# Autodesk Inventor assembly: NewChassis
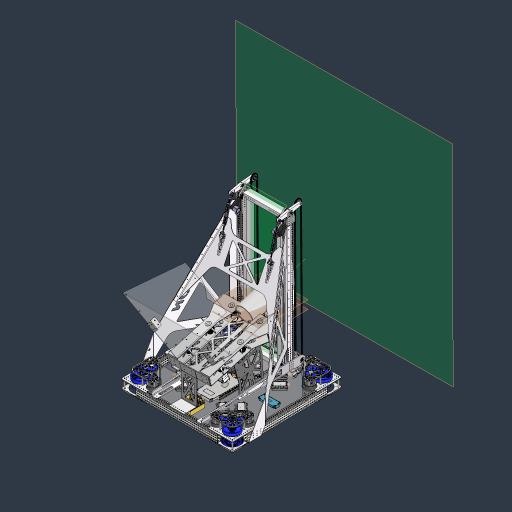
[picture p0: Inventor's stored thumbnail of the model, 512x512]
Saved by Autodesk Inventor 2024.3 (Build 283343000, 343)
## iProperties
ILogicPurgeVersion: 0.0.0.0
OnSaveVersion: 3.4.3.0
OnSaveAssembly: COREAutomationManager
Created: 2025-01-13
Part Number: NewChassis
Document SubType Name: Assembly
Designer: Marcus Tannini
Mfg Approved By: John.Thibert
Mass: 39455.4 g
Surface Area: 111693 cm^2
Volume: 16470.6 cm^3
Density: 2.3955 g/cm^3
ModelCat: Uncategorized
CN_MASS: 40.55
Author: Marcus Tannini
## Documents named in this file (60)
- D:\Inventor Projects\Poseidon V2\#Poseidon 2025.iam
- D:\Inventor Projects\Poseidon V2\ASSY,MK4i,Swerve_Module_INV.iam
- D:\Inventor Projects\Poseidon V2\MAXTube-2x1-Holes.ipt
- D:\Inventor Projects\Poseidon V2\BellyPanTop.ipt
- D:\Inventor Projects\Poseidon V2\BellyPanBot.ipt
- D:\Inventor Projects\Poseidon V2\BATTERY,12V.ipt
- D:\Inventor Projects\Poseidon V2\CONTROLS,MAIN_BREAKER.ipt
- D:\Inventor Projects\Poseidon V2\CONTROLS,MOTOR,NEO,550.ipt
- D:\Inventor Projects\Poseidon V2\CONTROLS,PDH.ipt
- D:\Inventor Projects\Poseidon V2\CONTROLS,PH.ipt
- D:\Inventor Projects\Poseidon V2\CONTROLS,ROBO_RIO.ipt
- D:\Inventor Projects\Poseidon V2\CONTROLS,SPARK_MAX.ipt
- D:\Inventor Projects\Poseidon V2\CONTROLS,VRM.ipt
- D:\Inventor Projects\Poseidon V2\COVER,SPARKMAX.ipt
- D:\Inventor Projects\Poseidon V2\ModifiedCase(IncludesPatterning).iam
- D:\Inventor Projects\Poseidon V2\PLATE,MOUNT,BATTERY,TOP.ipt
- D:\Inventor Projects\Poseidon V2\PLATE,MOUNT,BATTERY,BOT.ipt
- D:\Inventor Projects\Poseidon V2\MOUNT,STRAP,BATTERY.ipt
- D:\Inventor Projects\Poseidon V2\SPACER,SPROCKET,IDLER,ELEVATOR.ipt
- D:\Inventor Projects\Poseidon V2\22.ipt
- D:\Inventor Projects\Poseidon V2\PLATE,MOUNT,DRIVE,ELEVATOR.ipt
- D:\Inventor Projects\Poseidon V2\PLATE,BEARING,DRIVE,ELEVATOR.ipt
- D:\Inventor Projects\Poseidon V2\PURCHASED,HEX_BEARING.ipt
- D:\Inventor Projects\Poseidon V2\SHAFT,HEX,0.500in,DRIVE,ELEVATOR.ipt
- D:\Inventor Projects\Poseidon V2\PLATE,SIDE,BRACE,RIGHT,ELEVATOR.ipt
- D:\Inventor Projects\Poseidon V2\PLATE,SIDE,BRACE,LEFT,ELEVATOR.ipt
- D:\Inventor Projects\Poseidon V2\PLATE,TURNBUCKLE,TENSIONER,CHAIN.ipt
- D:\Inventor Projects\Poseidon V2\PLATE,BRACE,HORISONTAL,TOP,ELEVATOR.ipt
- D:\Inventor Projects\Poseidon V2\TURNBUCKLE,0.25IN_CLEVIS.iam
- D:\Inventor Projects\Poseidon V2\STAGE1,ELEVATOR.iam
- D:\Inventor Projects\Poseidon V2\ASSY,MAIN,ELEVATOR.iam
- D:\Inventor Projects\Poseidon V2\ANGLE,MOUNT,ELEVATOR.ipt
- D:\Inventor Projects\Poseidon V2\ANGLE,MOUNT,ELEVATOR,MIRR.ipt
- D:\Inventor Projects\Poseidon V2\FABRIC,BUMPERS.ipt
- D:\Inventor Projects\Poseidon V2\9293K119_Constant-Force Spring.ipt
- D:\Inventor Projects\Poseidon V2\MOUNT,SPRING,ELEVATOR.ipt
- D:\Inventor Projects\Poseidon V2\MOUNT,SPRING,ELEVATOR,MIRR.ipt
- D:\Inventor Projects\Poseidon V2\VersaPlanetary v2 Dual Stage 10_1 with RS 550 (1).iam
- D:\Inventor Projects\Poseidon V2\hopper_side_l.ipt
- D:\Inventor Projects\Poseidon V2\hopper_side_r.ipt
- D:\Inventor Projects\Poseidon V2\hopper_back.ipt
- D:\Inventor Projects\Poseidon V2\feeder_bottom_plate.ipt
- D:\Inventor Projects\Poseidon V2\hopper_side_bracket.ipt
- D:\Inventor Projects\Poseidon V2\feeder_guide_plate.ipt
- D:\Inventor Projects\Poseidon V2\am-5123 5IN 500IN Hex Bore Compliant Star.iam
- D:\Inventor Projects\Poseidon V2\feeder_guide_plate_MIR.ipt
- D:\Inventor Projects\Poseidon V2\feeder_front_support.ipt
- D:\Inventor Projects\Poseidon V2\Coral.ipt
- D:\Inventor Projects\Poseidon V2\coral_guide.ipt
- D:\Inventor Projects\Poseidon V2\coral_guide_MIR.ipt
- D:\Inventor Projects\Poseidon V2\hopper_back_support.ipt
- D:\Inventor Projects\Poseidon V2\feeder_side_support_r.ipt
- D:\Inventor Projects\Poseidon V2\feeder_side_support_l.ipt
- D:\Inventor Projects\Poseidon V2\feeder_middle_brace.ipt
- D:\Inventor Projects\Poseidon V2\2_1-2_hex_shaft.ipt
- D:\Inventor Projects\Poseidon V2\29t_hex\29t_hex.ipt
- D:\Inventor Projects\Poseidon V2\19t_hex\19t_hex.ipt
- D:\Inventor Projects\Poseidon V2\Bolt_Spacer.ipt
- D:\Inventor Projects\Poseidon V2\hopper_backboard.ipt
- D:\Inventor Projects\Poseidon V2\feeder_slide_plate.ipt
## Components (121 placed, 62 different names)
1. FABRIC,BUMPERS.ipt:1 — Flush:323, Mate:335, Mate:336
2. hopper_side_l:1 — Mate:496, Mate:497, Mate:498
3. hopper_side_r:1 — Mate:502, Mate:503, Mate:504
4. feeder_bottom_plate:1 — Angle:11, Mate:490, Mate:491, Mate:492, Mate:507, Mate:509, Mate:510, Mate:512, Mate:514, Mate:518, Flush:332, Mate:519, Mate:533, Mate:534, Mate:535, Angle:12, Flush:333, Mate:537, Flush:334, Mate:539, Flush:335, Mate:545, Mate:546, Mate:547, Flush:338, Flush:339, Mate:577, Mate:578, Mate:603, Mate:604, Mate:605, Insert:55, Insert:56, Insert:57, Insert:58, Mate:608, Mate:609, Mate:610, Mate:611, Mate:615, Mate:616, Mate:617
5. hopper_back:1 — Mate:490, Mate:491, Mate:492, Mate:493, Mate:494, Mate:495, Mate:499, Mate:500, Mate:501
6. hopper_side_bracket:1 — Mate:493, Mate:494, Mate:495, Mate:496, Mate:497, Mate:498
7. hopper_side_bracket:2 — Mate:499, Mate:500, Mate:501, Mate:502, Mate:503, Mate:504
8. feeder_guide_plate:1 — Mate:507, Mate:509, Insert:51, Insert:52, Mate:577
9. am-5123 5IN 500IN Hex Bore Compliant Star:2 [sub-assembly] — Mate:510, Mate:518, Flush:332, Flush:348
10. feeder_guide_plate_MIR:1 — Mate:512, Mate:514, Mate:520, Mate:578, Insert:53, Insert:54
11. feeder_front_support:1 — Mate:541, Mate:543, Mate:544
12. Coral:1 — Mate:519, Mate:520, Mate:521, Mate:522
13. CONTROLS,MOTOR,NEO,550:5
14. VersaPlanetary v2 Dual Stage 10_1 with RS 550 (1):3 [sub-assembly] — Mate:533, Mate:534, Mate:535, Mate:567, Mate:568
15. coral_guide:1 — Flush:333, Mate:537, Mate:540, Flush:335
16. coral_guide_MIR:1 — Flush:334, Mate:539, Mate:540
17. hopper_back_support:1 — Mate:545, Mate:546, Mate:547, Mate:548, Flush:336, Mate:549
18. feeder_side_support_r:1 — Flush:337, Flush:338, Flush:339, Mate:553, Mate:554, Mate:555, Mate:556, Mate:624, Mate:625, Mate:626
19. feeder_side_support_l:1 — Mate:550, Mate:551, Mate:552, Mate:627, Mate:628, Mate:629
20. feeder_middle_brace:1 — Mate:553, Mate:554, Mate:555
21. 2_1-2_hex_shaft:1 — Mate:557, Mate:558, Flush:340, Mate:561, Mate:562, Mate:565, Mate:566, Mate:569, Mate:570
22. PURCHASED,HEX_BEARING:3 — Insert:51, Mate:557, Mate:558, Flush:340, Mate:573
23. 2_1-2_hex_shaft:2 — Mate:563, Mate:564, Mate:571, Mate:572
24. PURCHASED,HEX_BEARING:4 — Insert:52, Mate:575
25. am-5123 5IN 500IN Hex Bore Compliant Star:3 [sub-assembly] — Mate:561, Mate:562, Mate:573, Mate:574
26. am-5123 5IN 500IN Hex Bore Compliant Star:4 [sub-assembly] — Mate:563, Mate:564, Mate:575
27. 29t_hex:1 — Mate:569, Mate:570, Flush:343, Mate:574, Mate:576
28. 19t_hex:1 — Mate:565, Mate:566, Flush:342, Mate:576
29. 19t_hex:2 — Mate:567, Mate:568, Flush:342, Flush:347
30. 29t_hex:2 — Mate:571, Mate:572, Flush:343
31. 2_1-2_hex_shaft:3
32. PURCHASED,HEX_BEARING:5 — Insert:53
33. am-5123 5IN 500IN Hex Bore Compliant Star:5 [sub-assembly]
34. 29t_hex:3 — Flush:346
35. 19t_hex:3
36. 2_1-2_hex_shaft:4 — Mate:597, Mate:598
37. PURCHASED,HEX_BEARING:6 — Insert:54
38. am-5123 5IN 500IN Hex Bore Compliant Star:6 [sub-assembly]
39. 29t_hex:4
40. 29t_hex:5 — Mate:597, Mate:598, Flush:346
41. am-5123 5IN 500IN Hex Bore Compliant Star:7 [sub-assembly] — Mate:606, Mate:607, Flush:348
42. CONTROLS,MOTOR,NEO,550:6
43. VersaPlanetary v2 Dual Stage 10_1 with RS 550 (1):4 [sub-assembly] — Mate:603, Mate:604, Mate:605, Mate:606, Mate:607
44. 19t_hex:4 — Flush:347
45. PURCHASED,HEX_BEARING:7 — Insert:58
46. PURCHASED,HEX_BEARING:8 — Insert:57
47. PURCHASED,HEX_BEARING:9 — Insert:56
48. PURCHASED,HEX_BEARING:10 — Insert:55
49. Bolt_Spacer:1 — Mate:608, Mate:609
50. Bolt_Spacer:2 — Mate:610, Mate:611
51. hopper_backboard:1 — Mate:612, Mate:613, Mate:614
52. feeder_slide_plate:1 — Mate:615, Mate:616, Mate:617
53. CONTROLS,SPARK_MAX:9 — Mate:626
54. COVER,SPARKMAX:9 — Mate:624, Mate:625
55. CONTROLS,SPARK_MAX:10 — Mate:629
56. COVER,SPARKMAX:10 — Mate:627, Mate:628
57. BellyPanBot.ipt:1 — Mate:66, Mate:353, Mate:354
58. BellyPanTop.ipt:1 — Mate:62, Mate:63, Mate:65, Mate:70, Mate:71, Mate:82, Mate:84, Insert:7, Insert:8, Insert:9, Insert:10, Insert:11, Insert:12, Insert:13, Insert:14, Insert:15, Insert:16, Insert:17, Insert:18, Insert:19, Insert:20, Insert:21, Insert:22, Mate:111, Mate:113, Mate:114, Mate:116, Mate:117, Mate:118, Mate:119, Mate:121, Mate:122, Mate:123, Mate:124, Mate:125, Mate:126, Mate:127, Mate:130, Insert:23, Insert:24, Mate:223, Mate:308, Mate:320, Mate:349, Mate:350, Angle:11, Mate:541, Mate:542, Mate:544, Mate:548, Flush:336, Mate:549
59. MAXTube-2x1-Holes.ipt:1 — Mate:1, Mate:2, Mate:3, Mate:4, Mate:5, Mate:15, Mate:115, Mate:272
60. MAXTube-2x1-Holes.ipt:2 — Mate:6, Mate:7, Mate:8, Mate:9, Mate:10, Mate:11, Mate:62, Flush:17, Mate:309, Mate:310, Mate:542, Mate:543
61. MAXTube-2x1-Holes.ipt:3 — Mate:19, Mate:20, Mate:21, Mate:66, Mate:114, Mate:312, Mate:313, Mate:336
62. MAXTube-2x1-Holes.ipt:4 — Mate:12, Mate:13, Mate:14, Mate:16, Mate:17, Mate:18, Mate:29, Mate:63, Mate:271, Mate:353, Mate:354
63. MOUNT,STRAP,BATTERY.ipt:1 — Mate:357, Mate:358, Mate:359
64. PLATE,MOUNT,BATTERY,BOT.ipt:1 — Mate:320, Mate:321, Mate:351, Mate:352
65. PLATE,MOUNT,BATTERY,TOP.ipt:1 — Mate:127, Mate:349, Mate:350, Mate:351, Mate:352, Mate:356, Mate:357, Mate:358, Mate:359
66. BATTERY,12V.ipt:1 — Mate:321, Mate:356
67. CONTROLS,MAIN_BREAKER.ipt:1 — Mate:82, Mate:111, Mate:116
68. CONTROLS,PDH.ipt:1 — Mate:113, Mate:117, Mate:118, Mate:119
69. CONTROLS,PH.ipt:1 — Insert:23, Insert:24
70. CONTROLS,ROBO_RIO.ipt:1 — Mate:124, Mate:125, Mate:126
71. CONTROLS,SPARK_MAX.ipt:1 — Mate:84, Mate:85, Mate:86, Mate:87
72. CONTROLS,VRM.ipt:1 — Mate:121, Mate:122, Mate:123
73. ModifiedCase(IncludesPatterning).iam:1 [sub-assembly] — Mate:130
74. ASSY,MK4i,Swerve_Module_INV.iam:1 [sub-assembly] — Mate:1, Mate:2, Mate:15
75. ASSY,MK4i,Swerve_Module_INV.iam:2 [sub-assembly] — Mate:3, Mate:4, Mate:5, Mate:6, Mate:7, Mate:8
76. ASSY,MK4i,Swerve_Module_INV.iam:3 [sub-assembly] — Mate:9, Mate:10, Mate:11, Mate:12, Mate:13, Mate:14
77. ASSY,MK4i,Swerve_Module_INV.iam:4 [sub-assembly] — Mate:16, Mate:17, Mate:18, Mate:19, Mate:20, Mate:21, Mate:67
78. CONTROLS,SPARK_MAX.ipt:2
79. CONTROLS,SPARK_MAX.ipt:3
80. CONTROLS,SPARK_MAX.ipt:4
81. CONTROLS,SPARK_MAX.ipt:5
82. CONTROLS,SPARK_MAX.ipt:6
83. CONTROLS,SPARK_MAX.ipt:7
84. CONTROLS,SPARK_MAX.ipt:8
85. COVER,SPARKMAX.ipt:1 — Mate:85, Mate:86, Mate:87, Insert:7, Insert:8
86. COVER,SPARKMAX.ipt:2 — Insert:9, Insert:10
87. COVER,SPARKMAX.ipt:3 — Insert:11, Insert:12
88. COVER,SPARKMAX.ipt:4 — Insert:13, Insert:14
89. COVER,SPARKMAX.ipt:5 — Insert:17, Insert:18
90. COVER,SPARKMAX.ipt:6 — Insert:15, Insert:16
91. COVER,SPARKMAX.ipt:7 — Insert:21, Insert:22
92. COVER,SPARKMAX.ipt:8 — Insert:19, Insert:20
93. 9293K119_Constant-Force Spring:1 — Mate:364, Mate:365
94. 9293K119_Constant-Force Spring:2 — Mate:370, Mate:371
95. MOUNT,SPRING,ELEVATOR:1 — Mate:363, Mate:362, Mate:364, Mate:365, Mate:366
96. MOUNT,SPRING,ELEVATOR,MIRR:1 — Mate:367, Mate:368, Mate:369, Mate:370, Mate:371
97. CONTROLS,MOTOR,NEO,550:3
98. VersaPlanetary v2 Dual Stage 10_1 with RS 550 (1):1 [sub-assembly] — Mate:472, Mate:473, Mate:474
99. CONTROLS,MOTOR,NEO,550:4
100. VersaPlanetary v2 Dual Stage 10_1 with RS 550 (1):2 [sub-assembly] — Mate:469, Mate:470, Mate:471
101. ASSY,MAIN,ELEVATOR.iam:1 [sub-assembly] — Mate:161, Mate:162, Flush:19, Mate:297, STAGE1 UPPER LIMIT, STAGE1 MAX, Mate:311, Mate:314, Mate:315, Mate:363, Mate:362, Mate:366, Mate:367, Mate:368, Mate:369
102. STAGE1,ELEVATOR.iam:1 [sub-assembly] — Flush:19, Mate:297, STAGE1 LOWER LIMIT, STAGE1 UPPER LIMIT, STAGE1 MIN, STAGE1 MAX, Mate:521
103. 22.ipt:1 — Mate:227, Angle:6
104. 22.ipt:2 — Mate:233, Angle:4, Flush:14
105. ANGLE,MOUNT,ELEVATOR.ipt:1 — Mate:65, Mate:70, Mate:71, Mate:161, Mate:162, Mate:224, STAGE1 LOWER LIMIT, STAGE1 MIN, Flush:337, Mate:556
106. ANGLE,MOUNT,ELEVATOR,MIRR.ipt:1 — Mate:308, Mate:309, Mate:310, Mate:311, Mate:312, Mate:313, Mate:314, Mate:315, Flush:329, Angle:12, Mate:550, Mate:551, Mate:552
107. PLATE,BEARING,DRIVE,ELEVATOR.ipt:1 — Mate:226, Mate:227, Mate:228, Mate:229, Insert:50
108. PLATE,BEARING,DRIVE,ELEVATOR.ipt:2 — Mate:230, Mate:231, Mate:232, Insert:49, Mate:233, Mate:234
109. PLATE,BRACE,HORISONTAL,TOP,ELEVATOR.ipt:1 — Mate:285, Mate:286, Mate:289, Mate:290, Mate:291, Mate:295, Mate:296, Mate:612, Mate:613, Mate:614
110. PLATE,MOUNT,DRIVE,ELEVATOR.ipt:1 — Mate:223, Mate:224, Mate:226, Mate:228, Mate:229, Mate:230, Mate:231, Mate:232, Flush:329, Mate:469, Mate:470, Mate:471, Mate:472, Mate:473, Mate:474
111. PLATE,SIDE,BRACE,LEFT,ELEVATOR.ipt:1 — Mate:271, Mate:289, Mate:290, Mate:291, Mate:335
112. PLATE,SIDE,BRACE,RIGHT,ELEVATOR.ipt:1 — Mate:272
113. PLATE,TURNBUCKLE,TENSIONER,CHAIN.ipt:1 — Mate:285, Mate:296
114. PLATE,TURNBUCKLE,TENSIONER,CHAIN.ipt:2 — Mate:286, Mate:295
115. PURCHASED,HEX_BEARING.ipt:1 — Insert:49, Angle:5
116. PURCHASED,HEX_BEARING.ipt:2 — Insert:50, Angle:7
117. SHAFT,HEX,0.500in,DRIVE,ELEVATOR.ipt:1 — Mate:234, Angle:4, Angle:5, Angle:6, Angle:7, Flush:14
118. SPACER,SPROCKET,IDLER,ELEVATOR.ipt:1
119. SPACER,SPROCKET,IDLER,ELEVATOR.ipt:2
120. TURNBUCKLE,0.25IN_CLEVIS.iam:1 [sub-assembly]
121. TURNBUCKLE,0.25IN_CLEVIS.iam:2 [sub-assembly]
## Relationships (339: Mate 275, Insert 32, Flush 26, Angle 6)
- Mate:1: MAXTube-2x1-Holes.ipt:1 ↔ ASSY,MK4i,Swerve_Module_INV.iam:1
- Mate:2: MAXTube-2x1-Holes.ipt:1 ↔ ASSY,MK4i,Swerve_Module_INV.iam:1
- Mate:3: MAXTube-2x1-Holes.ipt:1 ↔ ASSY,MK4i,Swerve_Module_INV.iam:2
- Mate:4: MAXTube-2x1-Holes.ipt:1 ↔ ASSY,MK4i,Swerve_Module_INV.iam:2
- Mate:5: MAXTube-2x1-Holes.ipt:1 ↔ ASSY,MK4i,Swerve_Module_INV.iam:2
- Mate:6: MAXTube-2x1-Holes.ipt:2 ↔ ASSY,MK4i,Swerve_Module_INV.iam:2
- Mate:7: MAXTube-2x1-Holes.ipt:2 ↔ ASSY,MK4i,Swerve_Module_INV.iam:2
- Mate:8: MAXTube-2x1-Holes.ipt:2 ↔ ASSY,MK4i,Swerve_Module_INV.iam:2
- Mate:9: MAXTube-2x1-Holes.ipt:2 ↔ ASSY,MK4i,Swerve_Module_INV.iam:3
- Mate:10: MAXTube-2x1-Holes.ipt:2 ↔ ASSY,MK4i,Swerve_Module_INV.iam:3
- Mate:11: MAXTube-2x1-Holes.ipt:2 ↔ ASSY,MK4i,Swerve_Module_INV.iam:3
- Mate:12: MAXTube-2x1-Holes.ipt:4 ↔ ASSY,MK4i,Swerve_Module_INV.iam:3
- Mate:13: MAXTube-2x1-Holes.ipt:4 ↔ ASSY,MK4i,Swerve_Module_INV.iam:3
- Mate:14: MAXTube-2x1-Holes.ipt:4 ↔ ASSY,MK4i,Swerve_Module_INV.iam:3
- Mate:15: MAXTube-2x1-Holes.ipt:1 ↔ ASSY,MK4i,Swerve_Module_INV.iam:1
- Mate:16: MAXTube-2x1-Holes.ipt:4 ↔ ASSY,MK4i,Swerve_Module_INV.iam:4
- Mate:17: MAXTube-2x1-Holes.ipt:4 ↔ ASSY,MK4i,Swerve_Module_INV.iam:4
- Mate:18: MAXTube-2x1-Holes.ipt:4 ↔ ASSY,MK4i,Swerve_Module_INV.iam:4
- Mate:19: MAXTube-2x1-Holes.ipt:3 ↔ ASSY,MK4i,Swerve_Module_INV.iam:4
- Mate:20: MAXTube-2x1-Holes.ipt:3 ↔ ASSY,MK4i,Swerve_Module_INV.iam:4
- Mate:21: MAXTube-2x1-Holes.ipt:3 ↔ ASSY,MK4i,Swerve_Module_INV.iam:4
- Mate:29 (-6.35 mm): MAXTube-2x1-Holes.ipt:4
- Mate:62: BellyPanTop.ipt:1 ↔ MAXTube-2x1-Holes.ipt:2
- Mate:63: BellyPanTop.ipt:1 ↔ MAXTube-2x1-Holes.ipt:4
- Mate:65: BellyPanTop.ipt:1 ↔ ANGLE,MOUNT,ELEVATOR.ipt:1
- Mate:66: BellyPanBot.ipt:1 ↔ MAXTube-2x1-Holes.ipt:3
- Mate:67 (35.56 mm): ASSY,MK4i,Swerve_Module_INV.iam:4
- Mate:70: BellyPanTop.ipt:1 ↔ ANGLE,MOUNT,ELEVATOR.ipt:1
- Mate:71: BellyPanTop.ipt:1 ↔ ANGLE,MOUNT,ELEVATOR.ipt:1
- Mate:321: PLATE,MOUNT,BATTERY,BOT.ipt:1 ↔ BATTERY,12V.ipt:1
- Mate:82: BellyPanTop.ipt:1 ↔ CONTROLS,MAIN_BREAKER.ipt:1
- Mate:84: BellyPanTop.ipt:1 ↔ CONTROLS,SPARK_MAX.ipt:1
- Mate:85: CONTROLS,SPARK_MAX.ipt:1 ↔ COVER,SPARKMAX.ipt:1
- Mate:86: CONTROLS,SPARK_MAX.ipt:1 ↔ COVER,SPARKMAX.ipt:1
- Mate:87: CONTROLS,SPARK_MAX.ipt:1 ↔ COVER,SPARKMAX.ipt:1
- Insert:7: BellyPanTop.ipt:1 ↔ COVER,SPARKMAX.ipt:1
- Insert:8: BellyPanTop.ipt:1 ↔ COVER,SPARKMAX.ipt:1
- [Mate]: CONTROLS,SPARK_MAX.ipt:2 ↔ COVER,SPARKMAX.ipt:2
- [Mate]: CONTROLS,SPARK_MAX.ipt:2 ↔ COVER,SPARKMAX.ipt:2
- [Mate]: CONTROLS,SPARK_MAX.ipt:2 ↔ COVER,SPARKMAX.ipt:2
- [Mate]: CONTROLS,SPARK_MAX.ipt:3 ↔ COVER,SPARKMAX.ipt:3
- [Mate]: CONTROLS,SPARK_MAX.ipt:3 ↔ COVER,SPARKMAX.ipt:3
- [Mate]: CONTROLS,SPARK_MAX.ipt:3 ↔ COVER,SPARKMAX.ipt:3
- [Mate]: CONTROLS,SPARK_MAX.ipt:4 ↔ COVER,SPARKMAX.ipt:4
- [Mate]: CONTROLS,SPARK_MAX.ipt:4 ↔ COVER,SPARKMAX.ipt:4
- [Mate]: CONTROLS,SPARK_MAX.ipt:4 ↔ COVER,SPARKMAX.ipt:4
- [Mate]: CONTROLS,SPARK_MAX.ipt:5 ↔ COVER,SPARKMAX.ipt:5
- [Mate]: CONTROLS,SPARK_MAX.ipt:5 ↔ COVER,SPARKMAX.ipt:5
- [Mate]: CONTROLS,SPARK_MAX.ipt:5 ↔ COVER,SPARKMAX.ipt:5
- [Mate]: CONTROLS,SPARK_MAX.ipt:6 ↔ COVER,SPARKMAX.ipt:6
- [Mate]: CONTROLS,SPARK_MAX.ipt:6 ↔ COVER,SPARKMAX.ipt:6
- [Mate]: CONTROLS,SPARK_MAX.ipt:6 ↔ COVER,SPARKMAX.ipt:6
- [Mate]: CONTROLS,SPARK_MAX.ipt:7 ↔ COVER,SPARKMAX.ipt:7
- [Mate]: CONTROLS,SPARK_MAX.ipt:7 ↔ COVER,SPARKMAX.ipt:7
- [Mate]: CONTROLS,SPARK_MAX.ipt:7 ↔ COVER,SPARKMAX.ipt:7
- [Mate]: CONTROLS,SPARK_MAX.ipt:8 ↔ COVER,SPARKMAX.ipt:8
- [Mate]: CONTROLS,SPARK_MAX.ipt:8 ↔ COVER,SPARKMAX.ipt:8
- [Mate]: CONTROLS,SPARK_MAX.ipt:8 ↔ COVER,SPARKMAX.ipt:8
- Insert:9: BellyPanTop.ipt:1 ↔ COVER,SPARKMAX.ipt:2
- Insert:10: BellyPanTop.ipt:1 ↔ COVER,SPARKMAX.ipt:2
- Insert:11: BellyPanTop.ipt:1 ↔ COVER,SPARKMAX.ipt:3
- Insert:12: BellyPanTop.ipt:1 ↔ COVER,SPARKMAX.ipt:3
- Insert:13: BellyPanTop.ipt:1 ↔ COVER,SPARKMAX.ipt:4
- Insert:14: BellyPanTop.ipt:1 ↔ COVER,SPARKMAX.ipt:4
- Insert:15: BellyPanTop.ipt:1 ↔ COVER,SPARKMAX.ipt:6
- Insert:16: BellyPanTop.ipt:1 ↔ COVER,SPARKMAX.ipt:6
- Insert:17: BellyPanTop.ipt:1 ↔ COVER,SPARKMAX.ipt:5
- Insert:18: BellyPanTop.ipt:1 ↔ COVER,SPARKMAX.ipt:5
- Insert:19: BellyPanTop.ipt:1 ↔ COVER,SPARKMAX.ipt:8
- Insert:20: BellyPanTop.ipt:1 ↔ COVER,SPARKMAX.ipt:8
- Insert:21: BellyPanTop.ipt:1 ↔ COVER,SPARKMAX.ipt:7
- Insert:22: BellyPanTop.ipt:1 ↔ COVER,SPARKMAX.ipt:7
- Mate:111: BellyPanTop.ipt:1 ↔ CONTROLS,MAIN_BREAKER.ipt:1
- Mate:113: BellyPanTop.ipt:1 ↔ CONTROLS,PDH.ipt:1
- Mate:114: BellyPanTop.ipt:1 ↔ MAXTube-2x1-Holes.ipt:3
- Mate:115 (-374.65 mm): MAXTube-2x1-Holes.ipt:1
- Mate:116 (0.254 mm): BellyPanTop.ipt:1 ↔ CONTROLS,MAIN_BREAKER.ipt:1
- Mate:117: BellyPanTop.ipt:1 ↔ CONTROLS,PDH.ipt:1
- Mate:118: BellyPanTop.ipt:1 ↔ CONTROLS,PDH.ipt:1
- Mate:119: BellyPanTop.ipt:1 ↔ CONTROLS,PDH.ipt:1
- Mate:121: BellyPanTop.ipt:1 ↔ CONTROLS,VRM.ipt:1
- Mate:122: BellyPanTop.ipt:1 ↔ CONTROLS,VRM.ipt:1
- Mate:123: BellyPanTop.ipt:1 ↔ CONTROLS,VRM.ipt:1
- Mate:124: BellyPanTop.ipt:1 ↔ CONTROLS,ROBO_RIO.ipt:1
- Mate:125: BellyPanTop.ipt:1 ↔ CONTROLS,ROBO_RIO.ipt:1
- Mate:126: BellyPanTop.ipt:1 ↔ CONTROLS,ROBO_RIO.ipt:1
- Mate:127: BellyPanTop.ipt:1 ↔ PLATE,MOUNT,BATTERY,TOP.ipt:1
- Mate:130: BellyPanTop.ipt:1 ↔ ModifiedCase(IncludesPatterning).iam:1
- Insert:23: BellyPanTop.ipt:1 ↔ CONTROLS,PH.ipt:1
- Insert:24: BellyPanTop.ipt:1 ↔ CONTROLS,PH.ipt:1
- Mate:161: ASSY,MAIN,ELEVATOR.iam:1 ↔ ANGLE,MOUNT,ELEVATOR.ipt:1
- Mate:162: ASSY,MAIN,ELEVATOR.iam:1 ↔ ANGLE,MOUNT,ELEVATOR.ipt:1
- [Mate]: ASSY,MAIN,ELEVATOR.iam:1 ↔ ANGLE,MOUNT,ELEVATOR.ipt:1
- [Insert]: ASSY,MAIN,ELEVATOR.iam:1 ↔ SPACER,SPROCKET,IDLER,ELEVATOR.ipt:1
- [Insert]: ASSY,MAIN,ELEVATOR.iam:1 ↔ SPACER,SPROCKET,IDLER,ELEVATOR.ipt:1
- [Flush]: ASSY,MAIN,ELEVATOR.iam:1 ↔ 22.ipt:1
- [Insert]: ASSY,MAIN,ELEVATOR.iam:1 ↔ SPACER,SPROCKET,IDLER,ELEVATOR.ipt:2
- [Insert]: ASSY,MAIN,ELEVATOR.iam:1 ↔ SPACER,SPROCKET,IDLER,ELEVATOR.ipt:2
- Mate:223: BellyPanTop.ipt:1 ↔ PLATE,MOUNT,DRIVE,ELEVATOR.ipt:1
- Mate:224: ANGLE,MOUNT,ELEVATOR.ipt:1 ↔ PLATE,MOUNT,DRIVE,ELEVATOR.ipt:1
- Mate:226: PLATE,BEARING,DRIVE,ELEVATOR.ipt:1 ↔ PLATE,MOUNT,DRIVE,ELEVATOR.ipt:1
- Mate:227: 22.ipt:1 ↔ PLATE,BEARING,DRIVE,ELEVATOR.ipt:1
- Mate:228: PLATE,BEARING,DRIVE,ELEVATOR.ipt:1 ↔ PLATE,MOUNT,DRIVE,ELEVATOR.ipt:1
- Mate:229: PLATE,BEARING,DRIVE,ELEVATOR.ipt:1 ↔ PLATE,MOUNT,DRIVE,ELEVATOR.ipt:1
- Mate:230: PLATE,BEARING,DRIVE,ELEVATOR.ipt:2 ↔ PLATE,MOUNT,DRIVE,ELEVATOR.ipt:1
- Mate:231: PLATE,BEARING,DRIVE,ELEVATOR.ipt:2 ↔ PLATE,MOUNT,DRIVE,ELEVATOR.ipt:1
- Mate:232: PLATE,BEARING,DRIVE,ELEVATOR.ipt:2 ↔ PLATE,MOUNT,DRIVE,ELEVATOR.ipt:1
- Insert:49: PLATE,BEARING,DRIVE,ELEVATOR.ipt:2 ↔ PURCHASED,HEX_BEARING.ipt:1
- Insert:50: PLATE,BEARING,DRIVE,ELEVATOR.ipt:1 ↔ PURCHASED,HEX_BEARING.ipt:2
- Mate:233: 22.ipt:2 ↔ PLATE,BEARING,DRIVE,ELEVATOR.ipt:2
- Mate:234: PLATE,BEARING,DRIVE,ELEVATOR.ipt:2 ↔ SHAFT,HEX,0.500in,DRIVE,ELEVATOR.ipt:1
- Angle:4 (0 deg): 22.ipt:2 ↔ SHAFT,HEX,0.500in,DRIVE,ELEVATOR.ipt:1
- Angle:5 (0 deg): PURCHASED,HEX_BEARING.ipt:1 ↔ SHAFT,HEX,0.500in,DRIVE,ELEVATOR.ipt:1
- Angle:6 (0 deg): 22.ipt:1 ↔ SHAFT,HEX,0.500in,DRIVE,ELEVATOR.ipt:1
- Angle:7 (0 deg): PURCHASED,HEX_BEARING.ipt:2 ↔ SHAFT,HEX,0.500in,DRIVE,ELEVATOR.ipt:1
- [Flush]: ASSY,MAIN,ELEVATOR.iam:1 ↔ 22.ipt:2
- [Mate]: ASSY,MAIN,ELEVATOR.iam:1 ↔ PLATE,SIDE,BRACE,LEFT,ELEVATOR.ipt:1
- [Mate]: ASSY,MAIN,ELEVATOR.iam:1 ↔ PLATE,SIDE,BRACE,LEFT,ELEVATOR.ipt:1
- [Mate]: ASSY,MAIN,ELEVATOR.iam:1 ↔ 22.ipt:1
- Flush:14 (-15.875 mm): 22.ipt:2 ↔ SHAFT,HEX,0.500in,DRIVE,ELEVATOR.ipt:1
- Flush:17 (457.2 mm): MAXTube-2x1-Holes.ipt:2
- [Mate]: ASSY,MAIN,ELEVATOR.iam:1 ↔ PLATE,SIDE,BRACE,LEFT,ELEVATOR.ipt:1
- [Mate]: ASSY,MAIN,ELEVATOR.iam:1 ↔ PLATE,SIDE,BRACE,RIGHT,ELEVATOR.ipt:1
- [Mate]: ASSY,MAIN,ELEVATOR.iam:1 ↔ PLATE,SIDE,BRACE,RIGHT,ELEVATOR.ipt:1
- [Mate]: ASSY,MAIN,ELEVATOR.iam:1 ↔ PLATE,SIDE,BRACE,RIGHT,ELEVATOR.ipt:1
- Mate:271: MAXTube-2x1-Holes.ipt:4 ↔ PLATE,SIDE,BRACE,LEFT,ELEVATOR.ipt:1
- Mate:272: MAXTube-2x1-Holes.ipt:1 ↔ PLATE,SIDE,BRACE,RIGHT,ELEVATOR.ipt:1
- [Mate]: ASSY,MAIN,ELEVATOR.iam:1 ↔ TURNBUCKLE,0.25IN_CLEVIS.iam:1
- [Mate]: ASSY,MAIN,ELEVATOR.iam:1 ↔ TURNBUCKLE,0.25IN_CLEVIS.iam:1
- [Mate]: ASSY,MAIN,ELEVATOR.iam:1 ↔ TURNBUCKLE,0.25IN_CLEVIS.iam:2
- [Mate]: ASSY,MAIN,ELEVATOR.iam:1 ↔ TURNBUCKLE,0.25IN_CLEVIS.iam:2
- Mate:285: PLATE,BRACE,HORISONTAL,TOP,ELEVATOR.ipt:1 ↔ PLATE,TURNBUCKLE,TENSIONER,CHAIN.ipt:1
- Mate:286: PLATE,BRACE,HORISONTAL,TOP,ELEVATOR.ipt:1 ↔ PLATE,TURNBUCKLE,TENSIONER,CHAIN.ipt:2
- Mate:289: PLATE,BRACE,HORISONTAL,TOP,ELEVATOR.ipt:1 ↔ PLATE,SIDE,BRACE,LEFT,ELEVATOR.ipt:1
- Mate:290: PLATE,BRACE,HORISONTAL,TOP,ELEVATOR.ipt:1 ↔ PLATE,SIDE,BRACE,LEFT,ELEVATOR.ipt:1
- Mate:291: PLATE,BRACE,HORISONTAL,TOP,ELEVATOR.ipt:1 ↔ PLATE,SIDE,BRACE,LEFT,ELEVATOR.ipt:1
- [Mate]: ASSY,MAIN,ELEVATOR.iam:1 ↔ 22.ipt:2
- Mate:295: PLATE,BRACE,HORISONTAL,TOP,ELEVATOR.ipt:1 ↔ PLATE,TURNBUCKLE,TENSIONER,CHAIN.ipt:2
- Mate:296: PLATE,BRACE,HORISONTAL,TOP,ELEVATOR.ipt:1 ↔ PLATE,TURNBUCKLE,TENSIONER,CHAIN.ipt:1
- Flush:19: ASSY,MAIN,ELEVATOR.iam:1 ↔ STAGE1,ELEVATOR.iam:1
- Mate:297: ASSY,MAIN,ELEVATOR.iam:1 ↔ STAGE1,ELEVATOR.iam:1
- STAGE1 LOWER LIMIT [Mate]: STAGE1,ELEVATOR.iam:1 ↔ ANGLE,MOUNT,ELEVATOR.ipt:1
- STAGE1 UPPER LIMIT [Mate]: ASSY,MAIN,ELEVATOR.iam:1 ↔ STAGE1,ELEVATOR.iam:1
- STAGE1 MIN [Mate]: STAGE1,ELEVATOR.iam:1 ↔ ANGLE,MOUNT,ELEVATOR.ipt:1
- STAGE1 MAX [Mate] (3.175 mm): ASSY,MAIN,ELEVATOR.iam:1 ↔ STAGE1,ELEVATOR.iam:1
- Mate:308: BellyPanTop.ipt:1 ↔ ANGLE,MOUNT,ELEVATOR,MIRR.ipt:1
- Mate:309: MAXTube-2x1-Holes.ipt:2 ↔ ANGLE,MOUNT,ELEVATOR,MIRR.ipt:1
- Mate:310: MAXTube-2x1-Holes.ipt:2 ↔ ANGLE,MOUNT,ELEVATOR,MIRR.ipt:1
- Mate:311: ASSY,MAIN,ELEVATOR.iam:1 ↔ ANGLE,MOUNT,ELEVATOR,MIRR.ipt:1
- Mate:312: MAXTube-2x1-Holes.ipt:3 ↔ ANGLE,MOUNT,ELEVATOR,MIRR.ipt:1
- Mate:313: MAXTube-2x1-Holes.ipt:3 ↔ ANGLE,MOUNT,ELEVATOR,MIRR.ipt:1
- Mate:314: ASSY,MAIN,ELEVATOR.iam:1 ↔ ANGLE,MOUNT,ELEVATOR,MIRR.ipt:1
- Mate:315: ASSY,MAIN,ELEVATOR.iam:1 ↔ ANGLE,MOUNT,ELEVATOR,MIRR.ipt:1
- Mate:320: BellyPanTop.ipt:1 ↔ PLATE,MOUNT,BATTERY,BOT.ipt:1
- Flush:323 (146.05 mm): FABRIC,BUMPERS.ipt:1
- Mate:335 (3.175 mm): FABRIC,BUMPERS.ipt:1 ↔ PLATE,SIDE,BRACE,LEFT,ELEVATOR.ipt:1
- Mate:336 (6.35 mm): FABRIC,BUMPERS.ipt:1 ↔ MAXTube-2x1-Holes.ipt:3
- Mate:349: BellyPanTop.ipt:1 ↔ PLATE,MOUNT,BATTERY,TOP.ipt:1
- Mate:350: BellyPanTop.ipt:1 ↔ PLATE,MOUNT,BATTERY,TOP.ipt:1
- Mate:351: PLATE,MOUNT,BATTERY,BOT.ipt:1 ↔ PLATE,MOUNT,BATTERY,TOP.ipt:1
- Mate:352: PLATE,MOUNT,BATTERY,BOT.ipt:1 ↔ PLATE,MOUNT,BATTERY,TOP.ipt:1
- Mate:353: BellyPanBot.ipt:1 ↔ MAXTube-2x1-Holes.ipt:4
- Mate:354: BellyPanBot.ipt:1 ↔ MAXTube-2x1-Holes.ipt:4
- Mate:356 (19.05 mm): PLATE,MOUNT,BATTERY,TOP.ipt:1 ↔ BATTERY,12V.ipt:1
- Mate:357: MOUNT,STRAP,BATTERY.ipt:1 ↔ PLATE,MOUNT,BATTERY,TOP.ipt:1
- Mate:358: MOUNT,STRAP,BATTERY.ipt:1 ↔ PLATE,MOUNT,BATTERY,TOP.ipt:1
- Mate:359: MOUNT,STRAP,BATTERY.ipt:1 ↔ PLATE,MOUNT,BATTERY,TOP.ipt:1
- Mate:363: MOUNT,SPRING,ELEVATOR:1 ↔ ASSY,MAIN,ELEVATOR.iam:1
- Mate:362: MOUNT,SPRING,ELEVATOR:1 ↔ ASSY,MAIN,ELEVATOR.iam:1
- Mate:364: 9293K119_Constant-Force Spring:1 ↔ MOUNT,SPRING,ELEVATOR:1
- Mate:365 (1.5875 mm): 9293K119_Constant-Force Spring:1 ↔ MOUNT,SPRING,ELEVATOR:1
- Mate:366: MOUNT,SPRING,ELEVATOR:1 ↔ ASSY,MAIN,ELEVATOR.iam:1
- Mate:367: MOUNT,SPRING,ELEVATOR,MIRR:1 ↔ ASSY,MAIN,ELEVATOR.iam:1
- Mate:368: MOUNT,SPRING,ELEVATOR,MIRR:1 ↔ ASSY,MAIN,ELEVATOR.iam:1
- Mate:369: MOUNT,SPRING,ELEVATOR,MIRR:1 ↔ ASSY,MAIN,ELEVATOR.iam:1
- Mate:370: 9293K119_Constant-Force Spring:2 ↔ MOUNT,SPRING,ELEVATOR,MIRR:1
- Mate:371 (1.5875 mm): 9293K119_Constant-Force Spring:2 ↔ MOUNT,SPRING,ELEVATOR,MIRR:1
- Flush:329: ANGLE,MOUNT,ELEVATOR,MIRR.ipt:1 ↔ PLATE,MOUNT,DRIVE,ELEVATOR.ipt:1
- [Mate]: CONTROLS,MOTOR,NEO,550:3 ↔ VersaPlanetary v2 Dual Stage 10_1 with RS 550 (1):1
- [Mate]: CONTROLS,MOTOR,NEO,550:3 ↔ VersaPlanetary v2 Dual Stage 10_1 with RS 550 (1):1
- [Mate]: CONTROLS,MOTOR,NEO,550:4 ↔ VersaPlanetary v2 Dual Stage 10_1 with RS 550 (1):2
- [Mate]: CONTROLS,MOTOR,NEO,550:4 ↔ VersaPlanetary v2 Dual Stage 10_1 with RS 550 (1):2
- Mate:469: VersaPlanetary v2 Dual Stage 10_1 with RS 550 (1):2 ↔ PLATE,MOUNT,DRIVE,ELEVATOR.ipt:1
- Mate:470: VersaPlanetary v2 Dual Stage 10_1 with RS 550 (1):2 ↔ PLATE,MOUNT,DRIVE,ELEVATOR.ipt:1
- Mate:471: VersaPlanetary v2 Dual Stage 10_1 with RS 550 (1):2 ↔ PLATE,MOUNT,DRIVE,ELEVATOR.ipt:1
- Mate:472: VersaPlanetary v2 Dual Stage 10_1 with RS 550 (1):1 ↔ PLATE,MOUNT,DRIVE,ELEVATOR.ipt:1
- Mate:473: VersaPlanetary v2 Dual Stage 10_1 with RS 550 (1):1 ↔ PLATE,MOUNT,DRIVE,ELEVATOR.ipt:1
- Mate:474: VersaPlanetary v2 Dual Stage 10_1 with RS 550 (1):1 ↔ PLATE,MOUNT,DRIVE,ELEVATOR.ipt:1
- Angle:11 (15 deg): feeder_bottom_plate:1 ↔ BellyPanTop.ipt:1
- Mate:490: feeder_bottom_plate:1 ↔ hopper_back:1
- Mate:491: feeder_bottom_plate:1 ↔ hopper_back:1
- Mate:492: feeder_bottom_plate:1 ↔ hopper_back:1
- Mate:493: hopper_back:1 ↔ hopper_side_bracket:1
- Mate:494: hopper_back:1 ↔ hopper_side_bracket:1
- Mate:495: hopper_back:1 ↔ hopper_side_bracket:1
- Mate:496: hopper_side_l:1 ↔ hopper_side_bracket:1
- Mate:497: hopper_side_l:1 ↔ hopper_side_bracket:1
- Mate:498: hopper_side_l:1 ↔ hopper_side_bracket:1
- Mate:499: hopper_back:1 ↔ hopper_side_bracket:2
- Mate:500: hopper_back:1 ↔ hopper_side_bracket:2
- Mate:501: hopper_back:1 ↔ hopper_side_bracket:2
- Mate:502: hopper_side_r:1 ↔ hopper_side_bracket:2
- Mate:503: hopper_side_r:1 ↔ hopper_side_bracket:2
- Mate:504: hopper_side_r:1 ↔ hopper_side_bracket:2
- Flush:330 (464.82 mm)
- Flush:331 (-57.15 mm)
- Mate:507: feeder_bottom_plate:1 ↔ feeder_guide_plate:1
- Mate:509 (55.5625 mm): feeder_bottom_plate:1 ↔ feeder_guide_plate:1
- Mate:510: feeder_bottom_plate:1 ↔ am-5123 5IN 500IN Hex Bore Compliant Star:2
- Mate:512: feeder_bottom_plate:1 ↔ feeder_guide_plate_MIR:1
- Mate:514 (55.5625 mm): feeder_bottom_plate:1 ↔ feeder_guide_plate_MIR:1
- Mate:518 (50.8 mm): feeder_bottom_plate:1 ↔ am-5123 5IN 500IN Hex Bore Compliant Star:2
- Flush:332 (27.8638 mm): feeder_bottom_plate:1 ↔ am-5123 5IN 500IN Hex Bore Compliant Star:2
- Mate:519 (57.15 mm): feeder_bottom_plate:1 ↔ Coral:1
- Mate:520 (58.7375 mm): feeder_guide_plate_MIR:1 ↔ Coral:1
- Mate:521: Coral:1 ↔ STAGE1,ELEVATOR.iam:1
- Mate:522: Coral:1
- [Mate]: CONTROLS,MOTOR,NEO,550:5 ↔ VersaPlanetary v2 Dual Stage 10_1 with RS 550 (1):3
- [Mate]: CONTROLS,MOTOR,NEO,550:5 ↔ VersaPlanetary v2 Dual Stage 10_1 with RS 550 (1):3
- Mate:533: feeder_bottom_plate:1 ↔ VersaPlanetary v2 Dual Stage 10_1 with RS 550 (1):3
- Mate:534: feeder_bottom_plate:1 ↔ VersaPlanetary v2 Dual Stage 10_1 with RS 550 (1):3
- Mate:535: feeder_bottom_plate:1 ↔ VersaPlanetary v2 Dual Stage 10_1 with RS 550 (1):3
- Angle:12 (180 deg): feeder_bottom_plate:1 ↔ ANGLE,MOUNT,ELEVATOR,MIRR.ipt:1
- Flush:333: feeder_bottom_plate:1 ↔ coral_guide:1
- Mate:537: feeder_bottom_plate:1 ↔ coral_guide:1
- Flush:334: feeder_bottom_plate:1 ↔ coral_guide_MIR:1
- Mate:539: feeder_bottom_plate:1 ↔ coral_guide_MIR:1
- Mate:540 (69.85 mm): coral_guide:1 ↔ coral_guide_MIR:1
- Flush:335 (11.1125 mm): feeder_bottom_plate:1 ↔ coral_guide:1
- Mate:541: feeder_front_support:1 ↔ BellyPanTop.ipt:1
- Mate:542: BellyPanTop.ipt:1 ↔ MAXTube-2x1-Holes.ipt:2
- Mate:543: feeder_front_support:1 ↔ MAXTube-2x1-Holes.ipt:2
- Mate:544: feeder_front_support:1 ↔ BellyPanTop.ipt:1
- Mate:545: feeder_bottom_plate:1 ↔ hopper_back_support:1
- Mate:546: feeder_bottom_plate:1 ↔ hopper_back_support:1
- Mate:547: feeder_bottom_plate:1 ↔ hopper_back_support:1
- Mate:548: hopper_back_support:1 ↔ BellyPanTop.ipt:1
- Flush:336: hopper_back_support:1 ↔ BellyPanTop.ipt:1
- Mate:549: hopper_back_support:1 ↔ BellyPanTop.ipt:1
- Flush:337: feeder_side_support_r:1 ↔ ANGLE,MOUNT,ELEVATOR.ipt:1
- Flush:338: feeder_bottom_plate:1 ↔ feeder_side_support_r:1
- Flush:339: feeder_bottom_plate:1 ↔ feeder_side_support_r:1
- Mate:550: feeder_side_support_l:1 ↔ ANGLE,MOUNT,ELEVATOR,MIRR.ipt:1
- Mate:551: feeder_side_support_l:1 ↔ ANGLE,MOUNT,ELEVATOR,MIRR.ipt:1
- Mate:552: feeder_side_support_l:1 ↔ ANGLE,MOUNT,ELEVATOR,MIRR.ipt:1
- Mate:553: feeder_side_support_r:1 ↔ feeder_middle_brace:1
- Mate:554: feeder_side_support_r:1 ↔ feeder_middle_brace:1
- Mate:555: feeder_side_support_r:1 ↔ feeder_middle_brace:1
- Mate:556: feeder_side_support_r:1 ↔ ANGLE,MOUNT,ELEVATOR.ipt:1
- Insert:51: feeder_guide_plate:1 ↔ PURCHASED,HEX_BEARING:3
- Mate:557: 2_1-2_hex_shaft:1 ↔ PURCHASED,HEX_BEARING:3
- Mate:558: 2_1-2_hex_shaft:1 ↔ PURCHASED,HEX_BEARING:3
- Flush:340: 2_1-2_hex_shaft:1 ↔ PURCHASED,HEX_BEARING:3
- [Mate]: 2_1-2_hex_shaft:2 ↔ PURCHASED,HEX_BEARING:4
- [Mate]: 2_1-2_hex_shaft:2 ↔ PURCHASED,HEX_BEARING:4
- [Flush]: 2_1-2_hex_shaft:2 ↔ PURCHASED,HEX_BEARING:4
- Insert:52: feeder_guide_plate:1 ↔ PURCHASED,HEX_BEARING:4
- Mate:561: 2_1-2_hex_shaft:1 ↔ am-5123 5IN 500IN Hex Bore Compliant Star:3
- Mate:562: 2_1-2_hex_shaft:1 ↔ am-5123 5IN 500IN Hex Bore Compliant Star:3
- Mate:563: 2_1-2_hex_shaft:2 ↔ am-5123 5IN 500IN Hex Bore Compliant Star:4
- Mate:564: 2_1-2_hex_shaft:2 ↔ am-5123 5IN 500IN Hex Bore Compliant Star:4
- Mate:565: 2_1-2_hex_shaft:1 ↔ 19t_hex:1
- Mate:566: 2_1-2_hex_shaft:1 ↔ 19t_hex:1
- Mate:567: VersaPlanetary v2 Dual Stage 10_1 with RS 550 (1):3 ↔ 19t_hex:2
- Mate:568: VersaPlanetary v2 Dual Stage 10_1 with RS 550 (1):3 ↔ 19t_hex:2
- Flush:342: 19t_hex:1 ↔ 19t_hex:2
- Mate:569: 2_1-2_hex_shaft:1 ↔ 29t_hex:1
- Mate:570: 2_1-2_hex_shaft:1 ↔ 29t_hex:1
- Mate:571: 2_1-2_hex_shaft:2 ↔ 29t_hex:2
- Mate:572: 2_1-2_hex_shaft:2 ↔ 29t_hex:2
- Flush:343: 29t_hex:1 ↔ 29t_hex:2
- Mate:573: PURCHASED,HEX_BEARING:3 ↔ am-5123 5IN 500IN Hex Bore Compliant Star:3
- Mate:574: am-5123 5IN 500IN Hex Bore Compliant Star:3 ↔ 29t_hex:1
- Mate:575: PURCHASED,HEX_BEARING:4 ↔ am-5123 5IN 500IN Hex Bore Compliant Star:4
- Mate:576: 29t_hex:1 ↔ 19t_hex:1
- Mate:577: feeder_bottom_plate:1 ↔ feeder_guide_plate:1
- Mate:578: feeder_bottom_plate:1 ↔ feeder_guide_plate_MIR:1
- [Mate]: 2_1-2_hex_shaft:3 ↔ PURCHASED,HEX_BEARING:5
- [Mate]: 2_1-2_hex_shaft:3 ↔ PURCHASED,HEX_BEARING:5
- [Flush]: 2_1-2_hex_shaft:3 ↔ PURCHASED,HEX_BEARING:5
- [Mate]: 2_1-2_hex_shaft:3 ↔ am-5123 5IN 500IN Hex Bore Compliant Star:5
- [Mate]: 2_1-2_hex_shaft:3 ↔ am-5123 5IN 500IN Hex Bore Compliant Star:5
- [Mate]: 2_1-2_hex_shaft:3 ↔ 19t_hex:3
- [Mate]: 2_1-2_hex_shaft:3 ↔ 19t_hex:3
- [Mate]: 2_1-2_hex_shaft:3 ↔ 29t_hex:3
- [Mate]: 2_1-2_hex_shaft:3 ↔ 29t_hex:3
- [Mate]: PURCHASED,HEX_BEARING:5 ↔ am-5123 5IN 500IN Hex Bore Compliant Star:5
- [Mate]: am-5123 5IN 500IN Hex Bore Compliant Star:5 ↔ 29t_hex:3
- [Mate]: 29t_hex:3 ↔ 19t_hex:3
- Insert:53: feeder_guide_plate_MIR:1 ↔ PURCHASED,HEX_BEARING:5
- [Mate]: 2_1-2_hex_shaft:4 ↔ PURCHASED,HEX_BEARING:6
- [Mate]: 2_1-2_hex_shaft:4 ↔ PURCHASED,HEX_BEARING:6
- [Flush]: 2_1-2_hex_shaft:4 ↔ PURCHASED,HEX_BEARING:6
- [Mate]: 2_1-2_hex_shaft:4 ↔ am-5123 5IN 500IN Hex Bore Compliant Star:6
- [Mate]: 2_1-2_hex_shaft:4 ↔ am-5123 5IN 500IN Hex Bore Compliant Star:6
- [Mate]: 2_1-2_hex_shaft:4 ↔ 29t_hex:4
- [Mate]: 2_1-2_hex_shaft:4 ↔ 29t_hex:4
- [Mate]: PURCHASED,HEX_BEARING:6 ↔ am-5123 5IN 500IN Hex Bore Compliant Star:6
- Insert:54: feeder_guide_plate_MIR:1 ↔ PURCHASED,HEX_BEARING:6
- Mate:597: 2_1-2_hex_shaft:4 ↔ 29t_hex:5
- Mate:598: 2_1-2_hex_shaft:4 ↔ 29t_hex:5
- Flush:346: 29t_hex:3 ↔ 29t_hex:5
- [Mate]: CONTROLS,MOTOR,NEO,550:6 ↔ VersaPlanetary v2 Dual Stage 10_1 with RS 550 (1):4
- [Mate]: CONTROLS,MOTOR,NEO,550:6 ↔ VersaPlanetary v2 Dual Stage 10_1 with RS 550 (1):4
- [Mate]: VersaPlanetary v2 Dual Stage 10_1 with RS 550 (1):4 ↔ 19t_hex:4
- [Mate]: VersaPlanetary v2 Dual Stage 10_1 with RS 550 (1):4 ↔ 19t_hex:4
- Mate:603: feeder_bottom_plate:1 ↔ VersaPlanetary v2 Dual Stage 10_1 with RS 550 (1):4
- Mate:604: feeder_bottom_plate:1 ↔ VersaPlanetary v2 Dual Stage 10_1 with RS 550 (1):4
- Mate:605: feeder_bottom_plate:1 ↔ VersaPlanetary v2 Dual Stage 10_1 with RS 550 (1):4
- Flush:347: 19t_hex:2 ↔ 19t_hex:4
- Mate:606: am-5123 5IN 500IN Hex Bore Compliant Star:7 ↔ VersaPlanetary v2 Dual Stage 10_1 with RS 550 (1):4
- Mate:607: am-5123 5IN 500IN Hex Bore Compliant Star:7 ↔ VersaPlanetary v2 Dual Stage 10_1 with RS 550 (1):4
- Flush:348: am-5123 5IN 500IN Hex Bore Compliant Star:2 ↔ am-5123 5IN 500IN Hex Bore Compliant Star:7
- Insert:55: feeder_bottom_plate:1 ↔ PURCHASED,HEX_BEARING:10
- Insert:56: feeder_bottom_plate:1 ↔ PURCHASED,HEX_BEARING:9
- Insert:57: feeder_bottom_plate:1 ↔ PURCHASED,HEX_BEARING:8
- Insert:58: feeder_bottom_plate:1 ↔ PURCHASED,HEX_BEARING:7
- Mate:608: feeder_bottom_plate:1 ↔ Bolt_Spacer:1
- Mate:609: feeder_bottom_plate:1 ↔ Bolt_Spacer:1
- Mate:610: feeder_bottom_plate:1 ↔ Bolt_Spacer:2
- Mate:611: feeder_bottom_plate:1 ↔ Bolt_Spacer:2
- Mate:612: hopper_backboard:1 ↔ PLATE,BRACE,HORISONTAL,TOP,ELEVATOR.ipt:1
- Mate:613: hopper_backboard:1 ↔ PLATE,BRACE,HORISONTAL,TOP,ELEVATOR.ipt:1
- Mate:614: hopper_backboard:1 ↔ PLATE,BRACE,HORISONTAL,TOP,ELEVATOR.ipt:1
- Mate:615: feeder_bottom_plate:1 ↔ feeder_slide_plate:1
- Mate:616: feeder_bottom_plate:1 ↔ feeder_slide_plate:1
- Mate:617: feeder_bottom_plate:1 ↔ feeder_slide_plate:1
- [Mate]: CONTROLS,SPARK_MAX:9 ↔ COVER,SPARKMAX:9
- [Mate]: CONTROLS,SPARK_MAX:9 ↔ COVER,SPARKMAX:9
- [Mate]: CONTROLS,SPARK_MAX:9 ↔ COVER,SPARKMAX:9
- [Mate]: CONTROLS,SPARK_MAX:10 ↔ COVER,SPARKMAX:10
- [Mate]: CONTROLS,SPARK_MAX:10 ↔ COVER,SPARKMAX:10
- [Mate]: CONTROLS,SPARK_MAX:10 ↔ COVER,SPARKMAX:10
- Mate:624: feeder_side_support_r:1 ↔ COVER,SPARKMAX:9
- Mate:625: feeder_side_support_r:1 ↔ COVER,SPARKMAX:9
- Mate:626: feeder_side_support_r:1 ↔ CONTROLS,SPARK_MAX:9
- Mate:627: feeder_side_support_l:1 ↔ COVER,SPARKMAX:10
- Mate:628: feeder_side_support_l:1 ↔ COVER,SPARKMAX:10
- Mate:629: feeder_side_support_l:1 ↔ CONTROLS,SPARK_MAX:10
## Named parameters: d160_d155 = 0 mm, d161_d156 = 0 mm, d162_d157 = 0 mm, d163_d155 = 0 mm, d164_d156 = 0 mm, d165_d157 = 0 mm, d166_d155 = 0 mm, d167_d156 = 0 mm, d168_d157 = 0 mm, d169_d155 = 0 mm, d170_d156 = 0 mm, d171_d157 = 0 mm, d172_d155 = 0 mm, d173_d156 = 0 mm, d174_d157 = 0 mm, d175_d155 = 0 mm, d176_d156 = 0 mm, d177_d157 = 0 mm, d178_d155 = 0 mm, d179_d156 = 0 mm, d180_d157 = 0 mm, d518_d513 = 0 mm, d875_d873 = 0 mm, d876_d874 = 0 mm, d967_d875_d873 = 0 mm, d968_d876_d874 = 0 mm, d1153_d967_d875_d873 = 0 mm, d1154_d968_d876_d874 = 0 mm, d1199_d1196 = 0 mm, d1200_d1197 = 0 mm, d1201_d1198 = 0 mm, d1224_d1196 = 0 mm, d1225_d1197 = 0 mm, d1226_d1198 = 0 mm, d1227_d1203 = 0 mm, d1228_d1204 = 0 mm, d1229_d1207 = 0 mm, d1230_d1208 = 0 mm, d1231_d1213 = 0 mm, d1232_d1214 = 0 mm, d1233_d1218 = 0 mm, d1234_d1219 = 0 mm, d1235_d1221 = 0 mm, d1237_d1199_d1196 = 0 mm, d1238_d1200_d1197 = 0 mm, d1239_d1201_d1198 = 0 mm, d1240_d1205 = 0 mm, d1241_d1206 = 0 mm, d1242_d1215 = 0 mm, d1243_d1216 = 0 mm, d1244_d1220 = 0 mm, d1249_d1153_d967_d875_d873 = 0 mm, d1250_d1154_d968_d876_d874 = 0 mm, d1251_d1209 = 0 mm, d1252_d1210 = 0 mm, d1274_d169_d155 = 0 mm, d1275_d170_d156 = 0 mm, d1276_d171_d157 = 0 mm, d1277_d169_d155 = 0 mm, d1278_d170_d156 = 0 mm, d1279_d171_d157 = 0 mm
